# Autodesk Inventor assembly: Intake Assembly
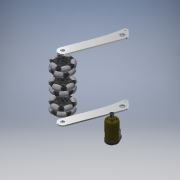
[picture p0: Inventor's stored thumbnail of the model, 180x180]
Saved by Autodesk Inventor 2019.4 (Build 234330000, 330)
## iProperties
Created: 2020-01-28
Part Number: Intake Assembly
Document SubType Name: Assembly
Designer: admin
Mass: 754.204 g
Surface Area: 2733.32 cm^2
Volume: 459.028 cm^3
Density: 1.64305 g/cm^3
Author: admin
## Documents named in this file (4)
- C:\Users\admin\Desktop\FRC 2020 Engineering\GitHub\7738-2020\Robot V2\Intake V2\Intake Assembly.iam
- C:\Users\admin\Desktop\FRC 2020 Engineering\GitHub\7738-2020\Robot V2\Intake V2\Intake Arm.ipt
- C:\Users\admin\Desktop\FRC 2020 Engineering\GitHub\7738-2020\Robot V2\Intake V2\Omni Wheel\3_25_Omni-Directional_Wheel_217-4775.iam
- C:\Users\admin\Desktop\FRC 2020 Engineering\GitHub\7738-2020\Robot V2\Turret\775\775pro_775pro_Connect_and_GT2_Pulley_217-6347 (1).iam
## Components (6 placed, 3 different names)
1. Intake Arm:1 — Mate:1, Mate:2, Mate:3, Mate:4, Mate:5, Mate:6, Mate:7, Mate:9
2. Intake Arm:2 — Mate:1, Mate:2, Mate:3, Mate:8
3. 3_25_Omni-Directional_Wheel_217-4775:1 [sub-assembly] — Mate:4
4. 3_25_Omni-Directional_Wheel_217-4775:2 [sub-assembly] — Mate:5
5. 3_25_Omni-Directional_Wheel_217-4775:3 [sub-assembly] — Mate:6
6. 775pro_775pro_Connect_and_GT2_Pulley_217-6347 (1):1 [sub-assembly] — Mate:9
## Relationships (9: Mate 9)
- Mate:1: Intake Arm:1 ↔ Intake Arm:2
- Mate:2: Intake Arm:1 ↔ Intake Arm:2
- Mate:3 (248.6 mm): Intake Arm:1 ↔ Intake Arm:2
- Mate:4: Intake Arm:1 ↔ 3_25_Omni-Directional_Wheel_217-4775:1
- Mate:5: Intake Arm:1 ↔ 3_25_Omni-Directional_Wheel_217-4775:2
- Mate:6: Intake Arm:1 ↔ 3_25_Omni-Directional_Wheel_217-4775:3
- Mate:7: Intake Arm:1
- Mate:8 (119.3 mm): Intake Arm:2
- Mate:9: Intake Arm:1 ↔ 775pro_775pro_Connect_and_GT2_Pulley_217-6347 (1):1
